# Autodesk Inventor assembly: Assembly1
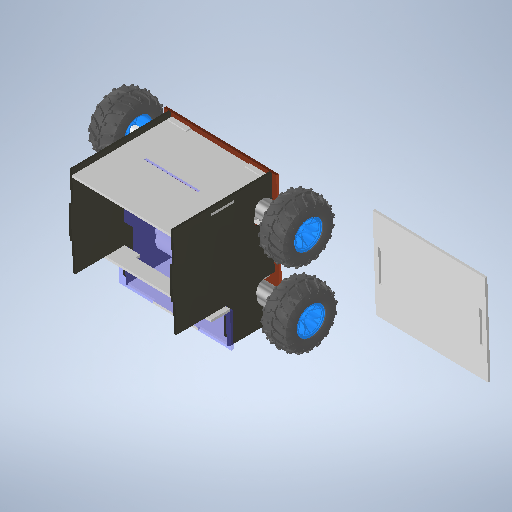
[picture p0: Inventor's stored thumbnail of the model, 512x512]
Saved by Autodesk Inventor 2025.3 (Build 293356030, 356C)
## iProperties
Created: 2026-06-26
Part Number: Assembly1
Document SubType Name: Assembly
Designer: user
Author: user
## Documents named in this file (12)
- C:\Docs\shcool\dojo\Design_2\Assembly1.iam
- C:\Docs\shcool\dojo\Design_2\hood.ipt
- C:\Docs\shcool\dojo\Design_2\side.ipt
- C:\Docs\shcool\dojo\Design_2\top.ipt
- C:\Docs\shcool\dojo\Design_2\back.ipt
- C:\Docs\shcool\dojo\Design_2\base_2.ipt
- C:\Docs\shcool\dojo\Design_1\Hub-12-Eixo6_aluminio.ipt
- C:\Docs\shcool\dojo\Design_3\motor_wheel\motor_dummy.ipt
- C:\Docs\shcool\dojo\Design_1\Spiked Rubber Wheel 120mm.ipt
- C:\Docs\shcool\dojo\Design_2\cover.ipt
- C:\Docs\shcool\dojo\Design_2\front.ipt
- C:\Docs\shcool\dojo\Design_2\U-bracket.ipt
## Components (24 placed, 11 different names)
1. hood:1 — Mate:78, Mate:79, Mate:80, Mate:81, Mate:82, Mate:83
2. side:1 — Mate:76, Mate:77, Mate:84, Mate:85
3. top:1
4. side:2 — Mate:78, Mate:79, Mate:98, Mate:99
5. back:1 — Mate:76, Mate:77
6. base_2:1 — Mate:57, Mate:84, Mate:85, Mate:87, Mate:90, Mate:91, Mate:92, Mate:95, Mate:98, Mate:99, Mate:100, Mate:101, Mate:102, Mate:103, Mate:104, Mate:105
7. motor_dummy:1 — Insert:3, Mate:63, Mate:68
8. Hub-12-Eixo6_aluminio:2 — Insert:3, Mate:29, Mate:30
9. Spiked Rubber Wheel 120mm:2 — Mate:29, Mate:30
10. cover:1 — Mate:80, Mate:81
11. motor_dummy:2 — Mate:65, Mate:69
12. Hub-12-Eixo6_aluminio:3
13. Spiked Rubber Wheel 120mm:3
14. motor_dummy:3 — Mate:62, Mate:67
15. Hub-12-Eixo6_aluminio:4
16. Spiked Rubber Wheel 120mm:4
17. motor_dummy:4 — Mate:64, Mate:66
18. Hub-12-Eixo6_aluminio:5
19. Spiked Rubber Wheel 120mm:5
20. U-bracket:1 — Mate:57, Mate:62, Mate:67, Mate:91, Mate:92
21. U-bracket:2 — Mate:65, Mate:69, Mate:95, Mate:102, Mate:103
22. U-bracket:3 — Mate:64, Mate:66, Mate:87, Mate:104, Mate:105
23. U-bracket:4 — Mate:63, Mate:68, Mate:90, Mate:100, Mate:101
24. front:1 — Mate:82, Mate:83
## Relationships (44: Mate 40, Insert 4)
- Insert:3: motor_dummy:1 ↔ Hub-12-Eixo6_aluminio:2
- Mate:29: Hub-12-Eixo6_aluminio:2 ↔ Spiked Rubber Wheel 120mm:2
- Mate:30: Hub-12-Eixo6_aluminio:2 ↔ Spiked Rubber Wheel 120mm:2
- [Insert]: motor_dummy:2 ↔ Hub-12-Eixo6_aluminio:3
- [Mate]: Hub-12-Eixo6_aluminio:3 ↔ Spiked Rubber Wheel 120mm:3
- [Mate]: Hub-12-Eixo6_aluminio:3 ↔ Spiked Rubber Wheel 120mm:3
- [Insert]: motor_dummy:3 ↔ Hub-12-Eixo6_aluminio:4
- [Mate]: Hub-12-Eixo6_aluminio:4 ↔ Spiked Rubber Wheel 120mm:4
- [Mate]: Hub-12-Eixo6_aluminio:4 ↔ Spiked Rubber Wheel 120mm:4
- [Insert]: motor_dummy:4 ↔ Hub-12-Eixo6_aluminio:5
- [Mate]: Hub-12-Eixo6_aluminio:5 ↔ Spiked Rubber Wheel 120mm:5
- [Mate]: Hub-12-Eixo6_aluminio:5 ↔ Spiked Rubber Wheel 120mm:5
- Mate:57: base_2:1 ↔ U-bracket:1
- Mate:62: motor_dummy:3 ↔ U-bracket:1
- Mate:63: motor_dummy:1 ↔ U-bracket:4
- Mate:64: motor_dummy:4 ↔ U-bracket:3
- Mate:65: motor_dummy:2 ↔ U-bracket:2
- Mate:66: motor_dummy:4 ↔ U-bracket:3
- Mate:67: motor_dummy:3 ↔ U-bracket:1
- Mate:68: motor_dummy:1 ↔ U-bracket:4
- Mate:69: motor_dummy:2 ↔ U-bracket:2
- Mate:76: side:1 ↔ back:1
- Mate:77: side:1 ↔ back:1
- Mate:78: hood:1 ↔ side:2
- Mate:79: hood:1 ↔ side:2
- Mate:80: hood:1 ↔ cover:1
- Mate:81: hood:1 ↔ cover:1
- Mate:82: hood:1 ↔ front:1
- Mate:83: hood:1 ↔ front:1
- Mate:84: side:1 ↔ base_2:1
- Mate:85: side:1 ↔ base_2:1
- Mate:87: base_2:1 ↔ U-bracket:3
- Mate:90: base_2:1 ↔ U-bracket:4
- Mate:91: base_2:1 ↔ U-bracket:1
- Mate:92: base_2:1 ↔ U-bracket:1
- Mate:95: base_2:1 ↔ U-bracket:2
- Mate:98: side:2 ↔ base_2:1
- Mate:99: side:2 ↔ base_2:1
- Mate:100: base_2:1 ↔ U-bracket:4
- Mate:101: base_2:1 ↔ U-bracket:4
- Mate:102: base_2:1 ↔ U-bracket:2
- Mate:103: base_2:1 ↔ U-bracket:2
- Mate:104: base_2:1 ↔ U-bracket:3
- Mate:105: base_2:1 ↔ U-bracket:3
## Named parameters: d85_d39 = 0 mm, d86_d47 = 0 mm, d87_d48 = 0 mm, d88_d39 = 0 mm, d89_d47 = 0 mm, d90_d48 = 0 mm, d91_d39 = 0 mm, d92_d47 = 0 mm, d93_d48 = 0 mm
